# Autodesk Inventor assembly: NewClaw
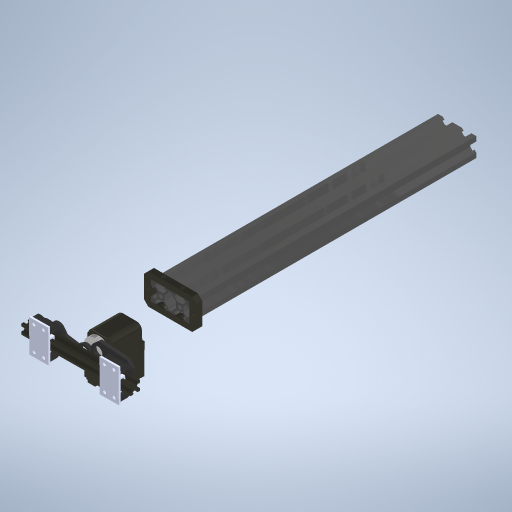
[picture p0: Inventor's stored thumbnail of the model, 512x512]
Saved by Autodesk Inventor 2024.3 (Build 283343000, 343)
## iProperties
Created: 2025-01-07
Part Number: NewClaw
Document SubType Name: Assembly
Designer: migue
Author: migue
## Documents named in this file (11)
- C:\Users\migue\Documents\GitHub\RobotCartesiano\DiseñoMecánico\Assemblies\NewClaw.iam
- C:\Users\migue\Documents\GitHub\RobotCartesiano\DiseñoMecánico\AcrylicPieces\ServoCarrier.ipt
- C:\Users\migue\Documents\GitHub\RobotCartesiano\DiseñoMecánico\Axis\AxisZ\MovingPlate\AP-ZClaw.ipt
- C:\Users\migue\Documents\GitHub\RobotCartesiano\DiseñoMecánico\Axis\AxisZ\MovingPlate\AP10x10.ipt
- C:\Users\migue\Documents\GitHub\RobotCartesiano\DiseñoMecánico\Axis\AxisZ\MovingPlate\MechanismArm.ipt
- C:\Users\migue\Documents\GitHub\RobotCartesiano\DiseñoMecánico\Motors\DynamixelAX12A\Pieces\AX12 middle.STEP.ipt
- C:\Users\migue\Documents\GitHub\RobotCartesiano\DiseñoMecánico\Motors\DynamixelAX12A\Pieces\AX12 Back.STEP.ipt
- C:\Users\migue\Documents\GitHub\RobotCartesiano\DiseñoMecánico\Motors\DynamixelAX12A\Pieces\AX12 Front.STEP.ipt
- C:\Users\migue\Documents\GitHub\RobotCartesiano\DiseñoMecánico\Motors\DynamixelAX12A\Pieces\Axel.STEP.ipt
- C:\Users\migue\Documents\GitHub\RobotCartesiano\DiseñoMecánico\Axis\AxisZ\MovingPlate\GripperSupport.ipt
- C:\Users\migue\Documents\GitHub\RobotCartesiano\DiseñoMecánico\Axis\AxisZ\MovingPlate\SliderPiece.ipt
## Components (13 placed, 10 different names)
1. ServoCarrier:1 — Mate:1, Flush:1, Mate:2
2. AP-ZClaw:1 — Mate:1, Flush:1, Mate:2
3. AP10x10:1 — Mate:17, Mate:18, Mate:19, Mate:20
4. MechanismArm:1 — Mate:7, Mate:8, Mate:23
5. MechanismArm:2 — Mate:9, Mate:10, Mate:21, Mate:22
6. Axel.STEP:1 — Mate:5, Mate:6, Mate:7, Mate:8, Mate:9, Mate:10
7. GripperSupport:4 — Mate:11, Mate:12, Mate:13, Mate:23
8. GripperSupport:5 — Mate:14, Mate:15, Mate:16, Mate:21, Mate:22
9. SliderPiece:1 — Mate:11, Mate:12, Mate:13, Mate:19, Mate:20
10. SliderPiece:2 — Mate:14, Mate:15, Mate:16, Mate:17, Mate:18
11. AX12 middle.STEP:1 — Mate:3, Flush:2, Flush:3, Flush:4, Mate:4, Flush:5
12. AX12 Back.STEP:1 — Mate:3, Flush:2, Flush:3
13. AX12 Front.STEP:1 — Flush:4, Mate:4, Flush:5, Mate:5, Mate:6
## Relationships (28: Mate 23, Flush 5)
- Mate:1: ServoCarrier:1 ↔ AP-ZClaw:1
- Flush:1: ServoCarrier:1 ↔ AP-ZClaw:1
- Mate:2: ServoCarrier:1 ↔ AP-ZClaw:1
- Mate:3: AX12 middle.STEP:1 ↔ AX12 Back.STEP:1
- Flush:2: AX12 middle.STEP:1 ↔ AX12 Back.STEP:1
- Flush:3: AX12 middle.STEP:1 ↔ AX12 Back.STEP:1
- Flush:4: AX12 middle.STEP:1 ↔ AX12 Front.STEP:1
- Mate:4: AX12 middle.STEP:1 ↔ AX12 Front.STEP:1
- Flush:5: AX12 middle.STEP:1 ↔ AX12 Front.STEP:1
- Mate:5: Axel.STEP:1 ↔ AX12 Front.STEP:1
- Mate:6: Axel.STEP:1 ↔ AX12 Front.STEP:1
- Mate:7: MechanismArm:1 ↔ Axel.STEP:1
- Mate:8: MechanismArm:1 ↔ Axel.STEP:1
- Mate:9: MechanismArm:2 ↔ Axel.STEP:1
- Mate:10: MechanismArm:2 ↔ Axel.STEP:1
- Mate:11: GripperSupport:4 ↔ SliderPiece:1
- Mate:12: GripperSupport:4 ↔ SliderPiece:1
- Mate:13: GripperSupport:4 ↔ SliderPiece:1
- Mate:14: GripperSupport:5 ↔ SliderPiece:2
- Mate:15: GripperSupport:5 ↔ SliderPiece:2
- Mate:16: GripperSupport:5 ↔ SliderPiece:2
- Mate:17: AP10x10:1 ↔ SliderPiece:2
- Mate:18: AP10x10:1 ↔ SliderPiece:2
- Mate:19: AP10x10:1 ↔ SliderPiece:1
- Mate:20: AP10x10:1 ↔ SliderPiece:1
- Mate:21: MechanismArm:2 ↔ GripperSupport:5
- Mate:22: MechanismArm:2 ↔ GripperSupport:5
- Mate:23: MechanismArm:1 ↔ GripperSupport:4
